# Autodesk Inventor assembly: Assembly_opentrons_microscope_slide_y_base
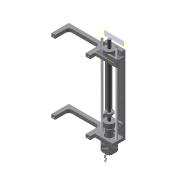
[picture p0: Inventor's stored thumbnail of the model, 180x180]
Saved by Autodesk Inventor 2019.4 (Build 234330000, 330)
## iProperties
Created: 2020-11-05
Part Number: Assembly_opentrons_microscope_slide_y_base
Document SubType Name: Assembly
Designer: diederichbenedict
Author: diederichbenedict
## Documents named in this file (5)
- C:\Users\diederichbenedict\Dropbox\Dokumente\Promotion\PROJECTS\OPENTRONS\INVENTOR\Assembly_opentrons_microscope_slide_y_base.iam
- C:\Users\diederichbenedict\Dropbox\Dokumente\Promotion\PROJECTS\OPENTRONS\INVENTOR\00_NEMA11.iam
- C:\Users\diederichbenedict\Dropbox\Dokumente\Promotion\PROJECTS\OPENTRONS\INVENTOR\02_Opentrons_Microscope_Base_v0.ipt
- C:\Users\diederichbenedict\Dropbox\Dokumente\Promotion\PROJECTS\OPENTRONS\INVENTOR\00_Thorlabs_Rod_200mm.ipt
- C:\Users\diederichbenedict\Dropbox\Dokumente\Promotion\PROJECTS\OPENTRONS\INVENTOR\Assembly_spindeldrive_350mm_2.iam
## Components (5 placed, 4 different names)
1. 00_NEMA11:1 [sub-assembly]
2. 02_Opentrons_Microscope_Base_v0:1
3. 00_Thorlabs_Rod_200mm:1
4. 00_Thorlabs_Rod_200mm:2
5. Assembly_spindeldrive_350mm_2:1 [sub-assembly]
## Relationships (5: Insert 3, Flush 2)
- [Insert]: 02_Opentrons_Microscope_Base_v0:1 ↔ 00_Thorlabs_Rod_200mm:2
- [Insert]: 02_Opentrons_Microscope_Base_v0:1 ↔ 00_Thorlabs_Rod_200mm:1
- [Insert] (3 mm): 00_NEMA11:1 ↔ Assembly_spindeldrive_350mm_2:1
- [Flush]: 02_Opentrons_Microscope_Base_v0:1 ↔ Assembly_spindeldrive_350mm_2:1
- [Flush] (2.5 mm): 02_Opentrons_Microscope_Base_v0:1 ↔ Assembly_spindeldrive_350mm_2:1
